# Autodesk Inventor assembly: Toolhead
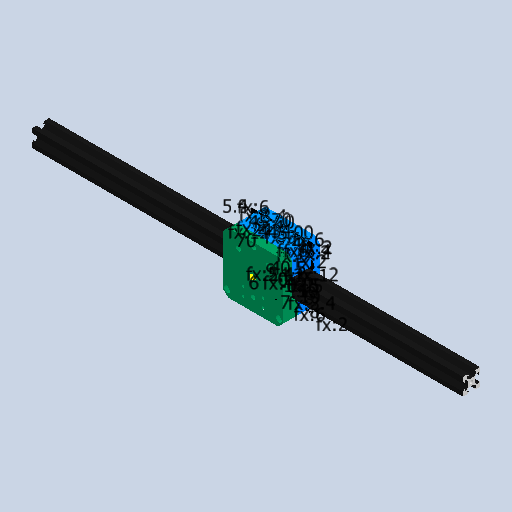
[picture p0: Inventor's stored thumbnail of the model, 512x512]
Saved by Autodesk Inventor 2025.1 (Build 291241000, 241)
## iProperties
Created: 2024-10-17
Part Number: Toolhead
Document SubType Name: Assembly
Designer: jerem
Author: jerem
## Documents named in this file (6)
- C:\Users\m_kni\OneDrive\Documents\GitHub\Perovskite-Automated-Synthesis-System\CAD\Gantry\Toolhead\Toolhead.iam
- C:\Users\m_kni\OneDrive\Documents\GitHub\Perovskite-Automated-Synthesis-System\CAD\Non 3D Printed Parts\Extrusion\V Extrustion 20x500mm.ipt
- C:\Users\m_kni\OneDrive\Documents\GitHub\Perovskite-Automated-Synthesis-System\CAD\Non 3D Printed Parts\Printer Wheel.ipt
- C:\Users\m_kni\OneDrive\Documents\GitHub\Perovskite-Automated-Synthesis-System\CAD\Gantry\Toolhead\Toolhead Base.ipt
- C:\Users\m_kni\OneDrive\Documents\GitHub\Perovskite-Automated-Synthesis-System\CAD\Gantry\Toolhead\Toolhead Cover.ipt
- C:\Users\m_kni\OneDrive\Documents\GitHub\Perovskite-Automated-Synthesis-System\CAD\Gantry\Toolhead\Belt Holders.ipt
## Components (8 placed, 5 different names)
1. V Extrustion 20x500mm:1 — Mate:7, Flush:1
2. Printer Wheel:1 — Mate:2, Mate:5, Mate:10
3. Printer Wheel:2 — Mate:3, Mate:6, Mate:7
4. Printer Wheel:3 — Mate:1, Mate:4, Mate:9
5. Toolhead Base:1 — Mate:1, Mate:2, Mate:3, Mate:4, Mate:5, Mate:6, Flush:1, Mate:11, Mate:12, Mate:13, Mate:14, Mate:15, Flush:2, Flush:3
6. Toolhead Cover:1 — Mate:9, Mate:10, Mate:11
7. Belt Holders:1 — Mate:12, Mate:15, Flush:2
8. Belt Holders:2 — Mate:13, Mate:14, Flush:3
## Relationships (17: Mate 14, Flush 3)
- Mate:1: Printer Wheel:3 ↔ Toolhead Base:1
- Mate:2: Printer Wheel:1 ↔ Toolhead Base:1
- Mate:3: Printer Wheel:2 ↔ Toolhead Base:1
- Mate:4: Printer Wheel:3 ↔ Toolhead Base:1
- Mate:5: Printer Wheel:1 ↔ Toolhead Base:1
- Mate:6: Printer Wheel:2 ↔ Toolhead Base:1
- Mate:7: V Extrustion 20x500mm:1 ↔ Printer Wheel:2
- Flush:1: V Extrustion 20x500mm:1 ↔ Toolhead Base:1
- Mate:9: Printer Wheel:3 ↔ Toolhead Cover:1
- Mate:10: Printer Wheel:1 ↔ Toolhead Cover:1
- Mate:11: Toolhead Base:1 ↔ Toolhead Cover:1
- Mate:12: Toolhead Base:1 ↔ Belt Holders:1
- Mate:13: Toolhead Base:1 ↔ Belt Holders:2
- Mate:14: Toolhead Base:1 ↔ Belt Holders:2
- Mate:15: Toolhead Base:1 ↔ Belt Holders:1
- Flush:2: Toolhead Base:1 ↔ Belt Holders:1
- Flush:3: Toolhead Base:1 ↔ Belt Holders:2
